# Autodesk Inventor assembly: A2017_T3_02
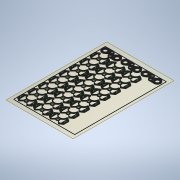
[picture p0: Inventor's stored thumbnail of the model, 180x180]
Saved by Autodesk Inventor 2022.3 (Build 263350000, 350)
## iProperties
Created: 2022-09-28
Part Number: A2017_T3_02
Document SubType Name: Assembly
Designer: Masato
Author: Masato
## Documents named in this file (4)
- C:\Users\Masato\Documents\Inventor\CIT Brains\SUSTAINA-OP - mod\Cam\A2017_T3\A2017_T3_02.iam
- C:\Users\Masato\Documents\Inventor\CIT Brains\SUSTAINA-OP - mod\Cam\DisposableBoard.ipt
- C:\Users\Masato\Documents\Inventor\CIT Brains\SUSTAINA-OP - mod\LowerBody\Slider_crank\Slider_crank_horn.ipt
- C:\Users\Masato\Documents\Inventor\CIT Brains\SUSTAINA-OP - mod\LowerBody\Leg_joint\Leg_joint_roll_frame.ipt
## Components (31 placed, 3 different names)
1. DisposableBoard:1 — フラッシュ:1, フラッシュ:2, フラッシュ:3, フラッシュ:4, Tangent:1, Flush:5, Flush:6, Tangent:2
2. Leg_joint_roll_frame:2 — Tangent:1, Flush:5, Mate:5
3. Leg_joint_roll_frame:3
4. Leg_joint_roll_frame:4
5. Leg_joint_roll_frame:5
6. Leg_joint_roll_frame:6
7. Leg_joint_roll_frame:7
8. Leg_joint_roll_frame:8
9. Leg_joint_roll_frame:9
10. Leg_joint_roll_frame:10
11. Leg_joint_roll_frame:11
12. Leg_joint_roll_frame:12
13. Leg_joint_roll_frame:13
14. Leg_joint_roll_frame:14
15. Leg_joint_roll_frame:15
16. Leg_joint_roll_frame:16
17. Leg_joint_roll_frame:17
18. Leg_joint_roll_frame:18
19. Leg_joint_roll_frame:19
20. Leg_joint_roll_frame:20
21. Leg_joint_roll_frame:21
22. Leg_joint_roll_frame:22
23. Leg_joint_roll_frame:23 — Mate:4
24. Leg_joint_roll_frame:24
25. Leg_joint_roll_frame:25
26. Slider_crank_horn:2 — Mate:1, Mate:2, Mate:4
27. Slider_crank_horn:1 — Flush:6, Mate:1, Mate:3, Tangent:2
28. Slider_crank_horn:3
29. Slider_crank_horn:4
30. Slider_crank_horn:5
31. Slider_crank_horn:6
## Component patterns: (24 elements, first: Leg_joint_roll_frame:2), (3 elements, first: Slider_crank_horn:2 + Slider_crank_horn:1)
## Relationships (13: Flush 6, Mate 5, Tangent 2)
- フラッシュ:1 [Flush]: DisposableBoard:1
- フラッシュ:2 [Flush]: DisposableBoard:1
- フラッシュ:3 [Flush]: DisposableBoard:1
- フラッシュ:4 [Flush]: DisposableBoard:1
- Tangent:1 (2 mm): DisposableBoard:1 ↔ Leg_joint_roll_frame:2
- Flush:5 (-2 mm): DisposableBoard:1 ↔ Leg_joint_roll_frame:2
- Flush:6 (-2.1 mm): DisposableBoard:1 ↔ Slider_crank_horn:1
- Mate:1 (2.1 mm): Slider_crank_horn:2 ↔ Slider_crank_horn:1
- Mate:2: Slider_crank_horn:2
- Mate:3: Slider_crank_horn:1
- Tangent:2 (2 mm): DisposableBoard:1 ↔ Slider_crank_horn:1
- Mate:4 (2.1 mm): Leg_joint_roll_frame:23 ↔ Slider_crank_horn:2
- Mate:5: Leg_joint_roll_frame:2
